# Autodesk Inventor assembly: Assembly5
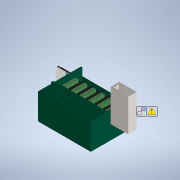
[picture p0: Inventor's stored thumbnail of the model, 180x180]
Saved by Autodesk Inventor 2020 (Build 240168000, 168)
## iProperties
Created: 2020-05-27
Part Number: Assembly5
Document SubType Name: Assembly
Designer: Gebruiker
Author: Gebruiker
## Documents named in this file (6)
- C:\Users\Gebruiker\Documents\GitHub\BeerMinder\3D-model\ControlBox\Assembly5.iam
- C:\Users\Gebruiker\Documents\GitHub\BeerMinder\3D-model\ControlBox\HY-DIV268N-5A.ipt
- C:\Users\Gebruiker\Documents\GitHub\BeerMinder\3D-model\ControlBox\controllbox_1.ipt
- C:\Users\Gebruiker\Documents\GitHub\BeerMinder\3D-model\ControlBox\LM2596_Buck_Converter.ipt
- C:\Users\Gebruiker\Documents\GitHub\BeerMinder\3D-model\ControlBox\ARDUINO DUE.ipt
- C:\Users\Gebruiker\Documents\GitHub\BeerMinder\3D-model\ControlBox\Power supply unit.iam
## Components (10 placed, 5 different names)
1. HY-DIV268N-5A:1 — Mate:1, Mate:3, Mate:4
2. HY-DIV268N-5A:2 — Mate:5, Mate:6, Mate:7
3. HY-DIV268N-5A:3 — Mate:8, Mate:9, Mate:10
4. HY-DIV268N-5A:4 — Mate:11, Mate:12, Mate:13
5. HY-DIV268N-5A:5 — Mate:14, Mate:15, Mate:16
6. HY-DIV268N-5A:6 — Mate:17, Mate:18, Mate:19
7. controllbox_1:1 — Mate:1, Mate:3, Mate:4, Mate:5, Mate:6, Mate:7, Mate:8, Mate:9, Mate:10, Mate:11, Mate:12, Mate:13, Mate:14, Mate:15, Mate:16, Mate:17, Mate:18, Mate:19, Mate:22, Mate:23, Mate:24
8. LM2596_Buck_Converter:1 — Mate:22, Mate:23
9. ARDUINO DUE:1
10. Power supply unit:1 [sub-assembly] — Mate:24
## Relationships (21: Mate 21)
- Mate:1: HY-DIV268N-5A:1 ↔ controllbox_1:1
- Mate:3: HY-DIV268N-5A:1 ↔ controllbox_1:1
- Mate:4: HY-DIV268N-5A:1 ↔ controllbox_1:1
- Mate:5: HY-DIV268N-5A:2 ↔ controllbox_1:1
- Mate:6: HY-DIV268N-5A:2 ↔ controllbox_1:1
- Mate:7: HY-DIV268N-5A:2 ↔ controllbox_1:1
- Mate:8: HY-DIV268N-5A:3 ↔ controllbox_1:1
- Mate:9: HY-DIV268N-5A:3 ↔ controllbox_1:1
- Mate:10: HY-DIV268N-5A:3 ↔ controllbox_1:1
- Mate:11: HY-DIV268N-5A:4 ↔ controllbox_1:1
- Mate:12: HY-DIV268N-5A:4 ↔ controllbox_1:1
- Mate:13: HY-DIV268N-5A:4 ↔ controllbox_1:1
- Mate:14: HY-DIV268N-5A:5 ↔ controllbox_1:1
- Mate:15: HY-DIV268N-5A:5 ↔ controllbox_1:1
- Mate:16: HY-DIV268N-5A:5 ↔ controllbox_1:1
- Mate:17: HY-DIV268N-5A:6 ↔ controllbox_1:1
- Mate:18: HY-DIV268N-5A:6 ↔ controllbox_1:1
- Mate:19: HY-DIV268N-5A:6 ↔ controllbox_1:1
- Mate:22: controllbox_1:1 ↔ LM2596_Buck_Converter:1
- Mate:23 (20 mm): controllbox_1:1 ↔ LM2596_Buck_Converter:1
- Mate:24: controllbox_1:1 ↔ Power supply unit:1
